# Autodesk Inventor assembly: vslot-belt-y
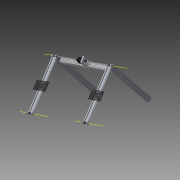
[picture p0: Inventor's stored thumbnail of the model, 180x180]
Saved by Autodesk Inventor 2015 (Build 190159000, 159)
## iProperties
Created: 2013-11-04
Part Number: vslot-belt-y
Document SubType Name: Assembly
Designer: Michael
Author: Michael
## Documents named in this file (7)
- C:\Users\Michael\Dropbox\autocad\openbuild\vslot-belt-y.iam
- C:\Users\Michael\Dropbox\autocad\openbuild\vslot-belt.iam
- C:\Users\Michael\Dropbox\autocad\openbuild\nema 17 with extended mount.iam
- C:\Users\Michael\Dropbox\autocad\openbuild\parts\280mm shaft.ipt
- C:\Users\Michael\Dropbox\autocad\openbuild\parts\STEP\Imported Components\5mm6mmCouplerS50TLCM13H05H06\5mm6mmCouplerS50TLCM13H05H06.ipt
- C:\Users\Michael\Dropbox\autocad\openbuild\parts\HFS5-4040-595.ipt
- C:\Users\Michael\Dropbox\autocad\openbuild\parts\HFS5-4040-530.ipt
## Components (10 placed, 6 different names)
1. vslot-belt:1 [sub-assembly] — Flush:1, Insert:7, Mate:6, Flush:7
2. vslot-belt:2 [sub-assembly] — Insert:2, Flush:1, Mate:1, Flush:2
3. nema 17 with extended mount:1 [sub-assembly] — Insert:5, Insert:6, Mate:5, Flush:5
4. 280mm shaft:1 — Insert:7, Mate:8
5. 280mm shaft:2 — Insert:2, Insert:3
6. 5mm6mmCouplerS50TLCM13H05H06:1 — Insert:5, Mate:8
7. 5mm6mmCouplerS50TLCM13H05H06:2 — Insert:3, Insert:6
8. HFS5-4040-595:1 — Mate:1, Flush:2, Mate:3, Flush:4
9. HFS5-4040-595:2 — Flush:6, Mate:6, Mate:7, Flush:7
10. HFS5-4040-530:1 — Mate:3, Flush:4, Mate:5, Flush:5, Flush:6, Mate:7
## Relationships (17: Flush 6, Mate 6, Insert 5)
- Insert:2 (-277 mm): vslot-belt:2 ↔ 280mm shaft:2
- Insert:3 (-5 mm): 280mm shaft:2 ↔ 5mm6mmCouplerS50TLCM13H05H06:2
- Insert:5 (-5 mm): nema 17 with extended mount:1 ↔ 5mm6mmCouplerS50TLCM13H05H06:1
- Insert:6 (-5 mm): nema 17 with extended mount:1 ↔ 5mm6mmCouplerS50TLCM13H05H06:2
- Flush:1: vslot-belt:1 ↔ vslot-belt:2
- Insert:7 (-3 mm): vslot-belt:1 ↔ 280mm shaft:1
- Mate:1: vslot-belt:2 ↔ HFS5-4040-595:1
- Flush:2: vslot-belt:2 ↔ HFS5-4040-595:1
- Mate:3: HFS5-4040-595:1 ↔ HFS5-4040-530:1
- Flush:4: HFS5-4040-595:1 ↔ HFS5-4040-530:1
- Mate:5: nema 17 with extended mount:1 ↔ HFS5-4040-530:1
- Flush:5: nema 17 with extended mount:1 ↔ HFS5-4040-530:1
- Flush:6: HFS5-4040-595:2 ↔ HFS5-4040-530:1
- Mate:6: vslot-belt:1 ↔ HFS5-4040-595:2
- Mate:7: HFS5-4040-595:2 ↔ HFS5-4040-530:1
- Flush:7: vslot-belt:1 ↔ HFS5-4040-595:2
- Mate:8: 280mm shaft:1 ↔ 5mm6mmCouplerS50TLCM13H05H06:1
